# Autodesk Inventor assembly: 8 Apparati V6
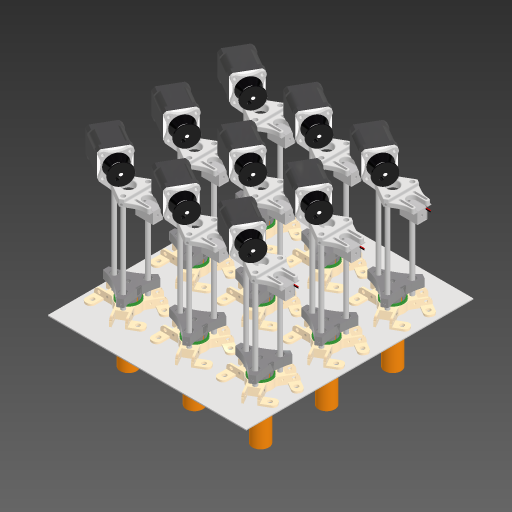
[picture p0: Inventor's stored thumbnail of the model, 512x512]
Saved by Autodesk Inventor 2024 (Build 280153000, 153)
## iProperties
Created: 2024-01-13
Part Number: 8 Apparati V6
Document SubType Name: Assembly
Designer: david
Author: david
## Documents named in this file (3)
- C:\Autodesk\ChalkBot Github\ChalkbotMechanical\Chalkbot1.0\Apparatus\V6\8 Apparati V6.iam
- C:\Autodesk\ChalkBot Github\ChalkbotMechanical\Chalkbot1.0\Chassis\V1\BasePlate.ipt
- C:\Autodesk\ChalkBot Github\ChalkbotMechanical\Chalkbot1.0\Apparatus\V6\Master Assembly V6.iam
## Components (10 placed, 2 different names)
1. BasePlate:1 — Mate:1, Mate:2
2. Master Assembly V6:1 [sub-assembly] — Mate:1, Mate:2
3. Master Assembly V6:2 [sub-assembly]
4. Master Assembly V6:3 [sub-assembly]
5. Master Assembly V6:4 [sub-assembly]
6. Master Assembly V6:5 [sub-assembly]
7. Master Assembly V6:6 [sub-assembly]
8. Master Assembly V6:7 [sub-assembly]
9. Master Assembly V6:8 [sub-assembly]
10. Master Assembly V6:9 [sub-assembly]
## Component patterns: (9 elements, first: Master Assembly V6:1)
## Relationships (2: Mate 2)
- Mate:1: BasePlate:1 ↔ Master Assembly V6:1
- Mate:2: BasePlate:1 ↔ Master Assembly V6:1
